# Autodesk Inventor assembly: Sistema Receptor de Senal
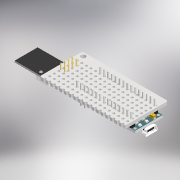
[picture p0: Inventor's stored thumbnail of the model, 180x180]
Saved by Autodesk Inventor 2021.4 (Build 254397000, 397)
## iProperties
Created: 2022-12-11
Part Number: Sistema Receptor de Senal
Document SubType Name: Assembly
Designer: crist
Author: crist
## Documents named in this file (4)
- C:\Users\crist\OneDrive - Escuela Superior Politécnica del Litoral\Escritorio\Archivos\Dron\Sistema Receptor de Senal.iam
- C:\Users\crist\OneDrive - Escuela Superior Politécnica del Litoral\Escritorio\Archivos\Dron\Modulo NRF24.ipt
- C:\Users\crist\OneDrive - Escuela Superior Politécnica del Litoral\Escritorio\Archivos\Dron\Arduino Nano.iam
- C:\Users\crist\OneDrive - Escuela Superior Politécnica del Litoral\Escritorio\Archivos\Dron\NRF24L1.ipt
## Components (3 placed, 3 different names)
1. Arduino Nano:1 [sub-assembly] — Rígido:1
2. Modulo NRF24:1 — Rígido:1, Rígido:2
3. NRF24L1:1 — Rígido:2
## Relationships (2: WeldJoint 2)
- Rígido:1 [WeldJoint]: Arduino Nano:1 ↔ Modulo NRF24:1
- Rígido:2 [WeldJoint]: Modulo NRF24:1 ↔ NRF24L1:1
